# Autodesk Inventor assembly: New_Case
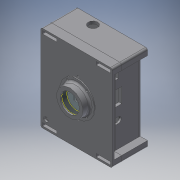
[picture p0: Inventor's stored thumbnail of the model, 180x180]
Saved by Autodesk Inventor 2017 (Build 210142000, 142)
## iProperties
Created: 2017-11-02
Part Number: New_Case
Document SubType Name: Assembly
Designer: P. Baesso
Author: P. Baesso
## Documents named in this file (9)
- E:\Rymapt_projects\Ethoscope\ethoscope_hardware\Assembled\New_Case.iam
- E:\Rymapt_projects\Ethoscope\ethoscope_hardware\core\RPi3\RPi3_ModelB.ipt
- E:\Rymapt_projects\Ethoscope\ethoscope_hardware\core_Rymapt\PiCase\lowerPiCase_small.ipt
- E:\Rymapt_projects\Ethoscope\ethoscope_hardware\core\RPi3\RasPi_Camera.ipt
- E:\Rymapt_projects\Ethoscope\ethoscope_hardware\Shield\Files\PCB_R2D2.iam
- E:\Rymapt_projects\Ethoscope\ethoscope_hardware\core_Rymapt\PiCase\upperPiCase_small.ipt
- E:\Rymapt_projects\Ethoscope\ethoscope_hardware\core_Rymapt\LightBox\sideWall_R3.ipt
- E:\Rymapt_projects\Ethoscope\ethoscope_hardware\extra\IRFilter\FB700-10-Step.ipt
- E:\Rymapt_projects\Ethoscope\ethoscope_hardware\extra\IRFilter\FilterHolder.ipt
## Components (9 placed, 8 different names)
1. RPi3_ModelB:1 — Angle:1, Angle:2, Flush:1, Flush:2, Mate:4, Flush:3, Mate:5, Flush:4
2. lowerPiCase_small:1 — Angle:1, Angle:2, Flush:1, Flush:2, Mate:4, Flush:6, Flush:7, Mate:6, Mate:7, Mate:8, Mate:9, Mate:10, Mate:11, Mate:12, Mate:13, Mate:14, Mate:15, Mate:17
3. RasPi_Camera:1 — Mate:13, Mate:14, Mate:15, Mate:16
4. PCB_R2D2:1 [sub-assembly] — Flush:3, Mate:5, Flush:4, Flush:5
5. upperPiCase_small:1 — Flush:6, Flush:7, Mate:6
6. sideWall_R3:1 — Mate:7, Mate:8, Mate:9
7. sideWall_R3:2 — Mate:10, Mate:11, Mate:12
8. FB700-10-Step:1 — Mate:16, Mate:17, Flush:8
9. FilterHolder:1 — Flush:8
## Relationships (24: Mate 14, Flush 8, Angle 2)
- Angle:1 (0 deg): RPi3_ModelB:1 ↔ lowerPiCase_small:1
- Angle:2 (0 deg): RPi3_ModelB:1 ↔ lowerPiCase_small:1
- Flush:1 (10.5 mm): RPi3_ModelB:1 ↔ lowerPiCase_small:1
- Flush:2: RPi3_ModelB:1 ↔ lowerPiCase_small:1
- Mate:4: RPi3_ModelB:1 ↔ lowerPiCase_small:1
- Flush:3: RPi3_ModelB:1 ↔ PCB_R2D2:1
- Mate:5 (1 mm): RPi3_ModelB:1 ↔ PCB_R2D2:1
- Flush:4: RPi3_ModelB:1 ↔ PCB_R2D2:1
- Flush:5 (1 mm): PCB_R2D2:1
- Flush:6: lowerPiCase_small:1 ↔ upperPiCase_small:1
- Flush:7: lowerPiCase_small:1 ↔ upperPiCase_small:1
- Mate:6: lowerPiCase_small:1 ↔ upperPiCase_small:1
- Mate:7: lowerPiCase_small:1 ↔ sideWall_R3:1
- Mate:8: lowerPiCase_small:1 ↔ sideWall_R3:1
- Mate:9: lowerPiCase_small:1 ↔ sideWall_R3:1
- Mate:10: lowerPiCase_small:1 ↔ sideWall_R3:2
- Mate:11: lowerPiCase_small:1 ↔ sideWall_R3:2
- Mate:12: lowerPiCase_small:1 ↔ sideWall_R3:2
- Mate:13: lowerPiCase_small:1 ↔ RasPi_Camera:1
- Mate:14: lowerPiCase_small:1 ↔ RasPi_Camera:1
- Mate:15: lowerPiCase_small:1 ↔ RasPi_Camera:1
- Mate:16: RasPi_Camera:1 ↔ FB700-10-Step:1
- Mate:17 (1 mm): lowerPiCase_small:1 ↔ FB700-10-Step:1
- Flush:8: FB700-10-Step:1 ↔ FilterHolder:1
